# Autodesk Inventor assembly: slideScrew
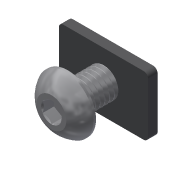
[picture p0: Inventor's stored thumbnail of the model, 180x180]
Saved by Autodesk Inventor 2017 (Build 210142000, 142)
## iProperties
Created: 2017-03-01
Part Number: slideScrew
Document SubType Name: Assembly
Designer: sawaiz
Author: sawaiz
## Documents named in this file (3)
- C:\Users\sawaiz\oneDrive\projects\sPhenixTileTestStand\hardware\slideScrew.iam
- C:\Users\sawaiz\oneDrive\projects\sPhenixTileTestStand\hardware\m5x10RoundHead.ipt
- C:\Users\sawaiz\oneDrive\projects\sPhenixTileTestStand\hardware\m5TNut.ipt
## Components (2 placed, 2 different names)
1. m5x10RoundHead:1 — Angle:1, Mate:1, Mate:2
2. m5TNut:1 — Angle:1, Mate:1, Mate:2
## Relationships (3: Mate 2, Angle 1)
- Angle:1 (180 deg): m5x10RoundHead:1 ↔ m5TNut:1
- Mate:1: m5x10RoundHead:1 ↔ m5TNut:1
- Mate:2 (6 mm): m5x10RoundHead:1 ↔ m5TNut:1
